# Autodesk Inventor assembly: Sessao_28_03_001_001
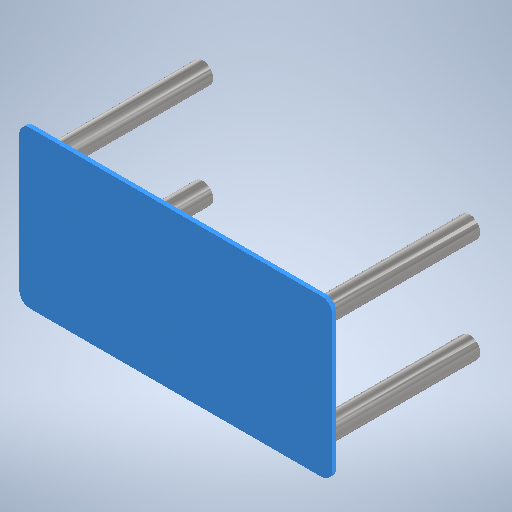
[picture p0: Inventor's stored thumbnail of the model, 512x512]
Saved by Autodesk Inventor 2026 (Build 300175000, 175)
## iProperties
Created: 2025-03-28
Part Number: Sessao_28_03_001_001
Document SubType Name: Assembly
Designer: Carlos Dias
Author: Carlos Dias
## Documents named in this file (3)
- C:\Users\Carlos Dias\Documents\Formação-TEARCI\UFCDs\5134 - Robótica _ Fundamentos\Material De Apoio\Sessao_28_03\Sessao_28_03_001_001.iam
- C:\Users\Carlos Dias\Documents\Formação-TEARCI\UFCDs\5134 - Robótica _ Fundamentos\Material De Apoio\Sessao_28_03\Sessao_28_03_001_001.ipt
- C:\Users\Carlos Dias\Documents\Formação-TEARCI\UFCDs\5134 - Robótica _ Fundamentos\Material De Apoio\Sessao_28_03\Sessao_28_03_002_001.ipt
## Components (5 placed, 2 different names)
1. Sessao_28_03_001_001:1 — Flush:1, Flush:2, Flush:3, Mate:1
2. Sessao_28_03_002_001:1 — Mate:3, Flush:6, Symmetry:1
3. Sessao_28_03_002_001:2 — Mate:4, Flush:7, Flush:8, Symmetry:1
4. Sessao_28_03_002_001:3 — Mate:2, Flush:6, Flush:8, Symmetry:2, Symmetry:3
5. Sessao_28_03_002_001:4 — Mate:1, Flush:4, Flush:5, Mate:2, Mate:3, Mate:4, Flush:7, Symmetry:2, Symmetry:3
## Relationships (15: Flush 8, Mate 4, Symmetry 3)
- Flush:1: Sessao_28_03_001_001:1
- Flush:2: Sessao_28_03_001_001:1
- Flush:3: Sessao_28_03_001_001:1
- Mate:1: Sessao_28_03_001_001:1 ↔ Sessao_28_03_002_001:4
- Flush:4 (640 mm): Sessao_28_03_002_001:4
- Flush:5 (250 mm): Sessao_28_03_002_001:4
- Mate:2: Sessao_28_03_002_001:3 ↔ Sessao_28_03_002_001:4
- Mate:3: Sessao_28_03_002_001:1 ↔ Sessao_28_03_002_001:4
- Mate:4: Sessao_28_03_002_001:2 ↔ Sessao_28_03_002_001:4
- Flush:6: Sessao_28_03_002_001:1 ↔ Sessao_28_03_002_001:3
- Flush:7: Sessao_28_03_002_001:2 ↔ Sessao_28_03_002_001:4
- Flush:8: Sessao_28_03_002_001:2 ↔ Sessao_28_03_002_001:3
- Symmetry:1: Sessao_28_03_002_001:1 ↔ Sessao_28_03_002_001:2
- Symmetry:2: Sessao_28_03_002_001:3 ↔ Sessao_28_03_002_001:4
- Symmetry:3: Sessao_28_03_002_001:3 ↔ Sessao_28_03_002_001:4
